# Autodesk Inventor assembly: 射出機構
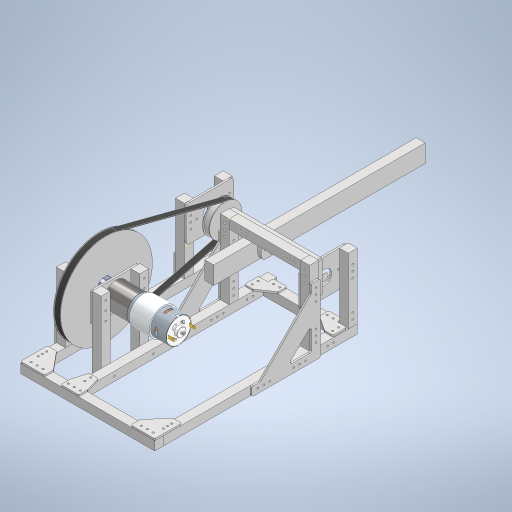
[picture p0: Inventor's stored thumbnail of the model, 512x512]
Saved by Autodesk Inventor 2023 (Build 270158000, 158)
## iProperties
Created: 2022-04-19
Part Number: 射出機構
Document SubType Name: Assembly
Designer: yuta
Author: yuta
## Documents named in this file (27)
- C:\Users\yuta\Documents\NHK\射出機構.iam
- C:\Users\yuta\Documents\NHK\RS775+gennsoku.iam
- C:\Users\yuta\Documents\NHK\射出_モーター固定1.ipt
- C:\Users\yuta\Documents\NHK\射出_type0.ipt
- C:\Users\yuta\Documents\NHK\射出_オムニ固定する.ipt
- C:\Users\yuta\Documents\NHK\射出_角柱1.ipt
- C:\Users\yuta\Documents\NHK\射出_角柱2.ipt
- C:\Users\yuta\Documents\NHK\射出_type1.ipt
- C:\Users\yuta\Documents\NHK\NHK.ipt
- C:\Users\yuta\Documents\NHK\射出_角柱3.ipt
- C:\Users\yuta\Documents\NHK\射出_角柱4.ipt
- C:\Users\yuta\Documents\NHK\射出_角柱5.ipt
- C:\Users\yuta\Documents\NHK\射出_角柱6.ipt
- C:\Users\yuta\Documents\NHK\射出_エンコーダー固定.ipt
- C:\Users\yuta\Documents\NHK\射出_固定1.ipt
- C:\Users\yuta\Documents\NHK\射出_軸.ipt
- C:\Users\yuta\Documents\NHK\射出_腕.ipt
- C:\Users\yuta\Documents\NHK\射出_角柱9.ipt
- C:\Users\yuta\Documents\NHK\射出_角柱10.ipt
- C:\Users\yuta\Documents\NHK\射出_角柱12.ipt
- C:\Users\yuta\Documents\NHK\射出_角柱11.ipt
- C:\Users\yuta\Documents\NHK\射出_受け身.ipt
- C:\Users\yuta\Documents\NHK\射出_固定2.ipt
- C:\Users\yuta\Documents\NHK\射出_固定3.ipt
- C:\Users\yuta\Documents\NHK\射出_固定4.ipt
- C:\Users\yuta\Documents\NHK\射出_固定5.ipt
- C:\Users\yuta\Documents\NHK\射出_腕固定.ipt
## Components (40 placed, 26 different names)
1. RS775+gennsoku:1 [sub-assembly] — メイト:1, メイト:2, メイト:3, メイト:4, メイト:6, メイト:16
2. 射出_モーター固定1:1 — メイト:1, メイト:2, メイト:9, メイト:10, メイト:11, メイト:12
3. 射出_オムニ固定する:1 — メイト:3, メイト:4, メイト:5
4. 射出_オムニ固定する:2 — メイト:7, メイト:8
5. 射出_type0:1 — メイト:5, メイト:6, メイト:7, メイト:8, メイト:15, メイト:17
6. 射出_角柱1:1 — メイト:9, メイト:10, メイト:13, メイト:14, メイト:47, メイト:48
7. 射出_角柱1:2 — メイト:11, メイト:12, メイト:46, メイト:48
8. 射出_角柱2:1 — メイト:13, メイト:14, フラッシュ:2, メイト:21, フラッシュ:5, フラッシュ:7, フラッシュ:8, メイト:46, メイト:47, フラッシュ:33, メイト:72, メイト:76, メイト:77
9. 射出_type1:1 — メイト:15, メイト:16, メイト:17, メイト:18, メイト:19
10. NHK:1 — メイト:18, メイト:19, メイト:35, メイト:36
11. 射出_角柱3:1 — フラッシュ:2, フラッシュ:3, メイト:20, フラッシュ:4, メイト:21, フラッシュ:5, フラッシュ:6, フラッシュ:8, メイト:22, フラッシュ:9, フラッシュ:10, メイト:67, メイト:68
12. 射出_角柱4:1 — フラッシュ:3, メイト:20, フラッシュ:4, フラッシュ:6, フラッシュ:7, メイト:37, フラッシュ:18, フラッシュ:19, メイト:53, フラッシュ:24, フラッシュ:25, メイト:58, フラッシュ:26, メイト:69, メイト:70
13. 射出_角柱5:1 — メイト:22, フラッシュ:9, フラッシュ:10, メイト:23, メイト:24, フラッシュ:11, メイト:25, フラッシュ:12, メイト:28, メイト:29, メイト:30, フラッシュ:15, フラッシュ:16, フラッシュ:17, メイト:31, メイト:66, メイト:74
14. 射出_角柱6:1 — メイト:25, メイト:26, フラッシュ:12, フラッシュ:14
15. 射出_角柱6:2 — メイト:23, メイト:24, フラッシュ:11, メイト:26, フラッシュ:13, メイト:27
16. 射出_エンコーダー固定:1 — フラッシュ:13, メイト:27, フラッシュ:14
17. 射出_固定1:2 — メイト:28, メイト:29
18. 射出_角柱6:3 — メイト:30, フラッシュ:15, フラッシュ:16, メイト:32, メイト:33, メイト:75
19. 射出_角柱6:4 — フラッシュ:17, メイト:31, メイト:32, メイト:34, フラッシュ:22
20. 射出_エンコーダー固定:2 — メイト:33, メイト:34, フラッシュ:22
21. 射出_オムニ固定する:3 — メイト:35, メイト:36
22. 射出_角柱6:5 — メイト:37, フラッシュ:18, フラッシュ:19
23. 射出_エンコーダー固定:3 — フラッシュ:23, メイト:45, メイト:55, フラッシュ:27
24. 射出_軸:1 — フラッシュ:23, メイト:45, メイト:54, メイト:79, メイト:81
25. 射出_角柱9:1 — メイト:53, フラッシュ:24, フラッシュ:25, メイト:71, メイト:73
26. 射出_腕:1 — メイト:54, メイト:55, メイト:78, メイト:80
27. 射出_角柱10:1 — メイト:58, フラッシュ:26, フラッシュ:27, メイト:59, フラッシュ:28, フラッシュ:29, メイト:62, メイト:63, メイト:64
28. 射出_角柱12:1 — メイト:59, フラッシュ:28, フラッシュ:29, メイト:60, フラッシュ:30, フラッシュ:31, メイト:61
29. 射出_角柱11:1 — メイト:60, フラッシュ:30, フラッシュ:31, メイト:65, フラッシュ:32, フラッシュ:34
30. 射出_受け身:1 — メイト:61, メイト:62, フラッシュ:34
31. 射出_固定2:2 — メイト:63, メイト:64
32. 射出_固定2:3 — メイト:65, フラッシュ:32, フラッシュ:33
33. 射出_固定3:1 — メイト:66, メイト:67
34. 射出_固定3:2 — メイト:68, メイト:69
35. 射出_固定4:1 — メイト:70, メイト:71
36. 射出_固定4:3 — メイト:72, メイト:73
37. 射出_固定1:3 — メイト:74, メイト:75
38. 射出_固定5:1 — メイト:76, メイト:77
39. 射出_腕固定:1 — メイト:78, メイト:79
40. 射出_腕固定:2 — メイト:80, メイト:81
## Relationships (99: Mate 68, Flush 31)
- メイト:1 [Mate]: RS775+gennsoku:1 ↔ 射出_モーター固定1:1
- メイト:2 [Mate]: RS775+gennsoku:1 ↔ 射出_モーター固定1:1
- メイト:3 [Mate]: RS775+gennsoku:1 ↔ 射出_オムニ固定する:1
- メイト:4 [Mate]: RS775+gennsoku:1 ↔ 射出_オムニ固定する:1
- メイト:5 [Mate]: 射出_オムニ固定する:1 ↔ 射出_type0:1
- メイト:6 [Mate]: RS775+gennsoku:1 ↔ 射出_type0:1
- メイト:7 [Mate]: 射出_オムニ固定する:2 ↔ 射出_type0:1
- メイト:8 [Mate]: 射出_オムニ固定する:2 ↔ 射出_type0:1
- メイト:9 [Mate]: 射出_モーター固定1:1 ↔ 射出_角柱1:1
- メイト:10 [Mate]: 射出_モーター固定1:1 ↔ 射出_角柱1:1
- メイト:11 [Mate]: 射出_モーター固定1:1 ↔ 射出_角柱1:2
- メイト:12 [Mate]: 射出_モーター固定1:1 ↔ 射出_角柱1:2
- メイト:13 [Mate]: 射出_角柱1:1 ↔ 射出_角柱2:1
- メイト:14 [Mate]: 射出_角柱1:1 ↔ 射出_角柱2:1
- メイト:15 [Mate]: 射出_type0:1 ↔ 射出_type1:1
- メイト:16 [Mate]: RS775+gennsoku:1 ↔ 射出_type1:1
- メイト:17 [Mate]: 射出_type0:1 ↔ 射出_type1:1
- メイト:18 [Mate]: 射出_type1:1 ↔ NHK:1
- メイト:19 [Mate]: 射出_type1:1 ↔ NHK:1
- フラッシュ:2 [Flush]: 射出_角柱2:1 ↔ 射出_角柱3:1
- フラッシュ:3 [Flush]: 射出_角柱3:1 ↔ 射出_角柱4:1
- メイト:20 [Mate]: 射出_角柱3:1 ↔ 射出_角柱4:1
- フラッシュ:4 [Flush]: 射出_角柱3:1 ↔ 射出_角柱4:1
- メイト:21 [Mate]: 射出_角柱2:1 ↔ 射出_角柱3:1
- フラッシュ:5 [Flush]: 射出_角柱2:1 ↔ 射出_角柱3:1
- フラッシュ:6 [Flush]: 射出_角柱3:1 ↔ 射出_角柱4:1
- フラッシュ:7 [Flush]: 射出_角柱2:1 ↔ 射出_角柱4:1
- フラッシュ:8 [Flush] (75 mm): 射出_角柱2:1 ↔ 射出_角柱3:1
- メイト:22 [Mate]: 射出_角柱3:1 ↔ 射出_角柱5:1
- フラッシュ:9 [Flush]: 射出_角柱3:1 ↔ 射出_角柱5:1
- フラッシュ:10 [Flush]: 射出_角柱3:1 ↔ 射出_角柱5:1
- メイト:23 [Mate]: 射出_角柱5:1 ↔ 射出_角柱6:2
- メイト:24 [Mate] (-60 mm): 射出_角柱5:1 ↔ 射出_角柱6:2
- フラッシュ:11 [Flush]: 射出_角柱5:1 ↔ 射出_角柱6:2
- メイト:25 [Mate]: 射出_角柱5:1 ↔ 射出_角柱6:1
- メイト:26 [Mate] (50 mm): 射出_角柱6:1 ↔ 射出_角柱6:2
- フラッシュ:12 [Flush]: 射出_角柱5:1 ↔ 射出_角柱6:1
- フラッシュ:13 [Flush]: 射出_角柱6:2 ↔ 射出_エンコーダー固定:1
- メイト:27 [Mate]: 射出_角柱6:2 ↔ 射出_エンコーダー固定:1
- フラッシュ:14 [Flush]: 射出_角柱6:1 ↔ 射出_エンコーダー固定:1
- メイト:28 [Mate]: 射出_角柱5:1 ↔ 射出_固定1:2
- メイト:29 [Mate]: 射出_角柱5:1 ↔ 射出_固定1:2
- メイト:30 [Mate]: 射出_角柱5:1 ↔ 射出_角柱6:3
- フラッシュ:15 [Flush]: 射出_角柱5:1 ↔ 射出_角柱6:3
- フラッシュ:16 [Flush]: 射出_角柱5:1 ↔ 射出_角柱6:3
- フラッシュ:17 [Flush]: 射出_角柱5:1 ↔ 射出_角柱6:4
- メイト:31 [Mate]: 射出_角柱5:1 ↔ 射出_角柱6:4
- メイト:32 [Mate] (50 mm): 射出_角柱6:3 ↔ 射出_角柱6:4
- メイト:33 [Mate]: 射出_角柱6:3 ↔ 射出_エンコーダー固定:2
- メイト:34 [Mate]: 射出_角柱6:4 ↔ 射出_エンコーダー固定:2
- メイト:35 [Mate]: NHK:1 ↔ 射出_オムニ固定する:3
- メイト:36 [Mate]: NHK:1 ↔ 射出_オムニ固定する:3
- メイト:37 [Mate]: 射出_角柱4:1 ↔ 射出_角柱6:5
- フラッシュ:18 [Flush]: 射出_角柱4:1 ↔ 射出_角柱6:5
- フラッシュ:19 [Flush]: 射出_角柱4:1 ↔ 射出_角柱6:5
- フラッシュ:22 [Flush]: 射出_角柱6:4 ↔ 射出_エンコーダー固定:2
- フラッシュ:23 [Flush]: 射出_エンコーダー固定:3 ↔ 射出_軸:1
- メイト:45 [Mate]: 射出_エンコーダー固定:3 ↔ 射出_軸:1
- メイト:46 [Mate]: 射出_角柱1:2 ↔ 射出_角柱2:1
- メイト:47 [Mate]: 射出_角柱1:1 ↔ 射出_角柱2:1
- メイト:48 [Mate] (50 mm): 射出_角柱1:1 ↔ 射出_角柱1:2
- メイト:53 [Mate]: 射出_角柱4:1 ↔ 射出_角柱9:1
- フラッシュ:24 [Flush] (8 mm): 射出_角柱4:1 ↔ 射出_角柱9:1
- フラッシュ:25 [Flush]: 射出_角柱4:1 ↔ 射出_角柱9:1
- メイト:54 [Mate]: 射出_軸:1 ↔ 射出_腕:1
- メイト:55 [Mate] (93 mm): 射出_エンコーダー固定:3 ↔ 射出_腕:1
- メイト:58 [Mate]: 射出_角柱4:1 ↔ 射出_角柱10:1
- フラッシュ:26 [Flush]: 射出_角柱4:1 ↔ 射出_角柱10:1
- フラッシュ:27 [Flush]: 射出_エンコーダー固定:3 ↔ 射出_角柱10:1
- メイト:59 [Mate]: 射出_角柱10:1 ↔ 射出_角柱12:1
- フラッシュ:28 [Flush]: 射出_角柱10:1 ↔ 射出_角柱12:1
- フラッシュ:29 [Flush]: 射出_角柱10:1 ↔ 射出_角柱12:1
- メイト:60 [Mate]: 射出_角柱12:1 ↔ 射出_角柱11:1
- フラッシュ:30 [Flush]: 射出_角柱12:1 ↔ 射出_角柱11:1
- フラッシュ:31 [Flush]: 射出_角柱12:1 ↔ 射出_角柱11:1
- メイト:61 [Mate]: 射出_角柱12:1 ↔ 射出_受け身:1
- メイト:62 [Mate]: 射出_角柱10:1 ↔ 射出_受け身:1
- メイト:63 [Mate]: 射出_角柱10:1 ↔ 射出_固定2:2
- メイト:64 [Mate]: 射出_角柱10:1 ↔ 射出_固定2:2
- メイト:65 [Mate]: 射出_角柱11:1 ↔ 射出_固定2:3
- フラッシュ:32 [Flush]: 射出_角柱11:1 ↔ 射出_固定2:3
- フラッシュ:33 [Flush]: 射出_角柱2:1 ↔ 射出_固定2:3
- メイト:66 [Mate]: 射出_角柱5:1 ↔ 射出_固定3:1
- メイト:67 [Mate]: 射出_角柱3:1 ↔ 射出_固定3:1
- メイト:68 [Mate]: 射出_角柱3:1 ↔ 射出_固定3:2
- メイト:69 [Mate]: 射出_角柱4:1 ↔ 射出_固定3:2
- メイト:70 [Mate]: 射出_角柱4:1 ↔ 射出_固定4:1
- メイト:71 [Mate]: 射出_角柱9:1 ↔ 射出_固定4:1
- メイト:72 [Mate]: 射出_角柱2:1 ↔ 射出_固定4:3
- メイト:73 [Mate]: 射出_角柱9:1 ↔ 射出_固定4:3
- メイト:74 [Mate]: 射出_角柱5:1 ↔ 射出_固定1:3
- メイト:75 [Mate]: 射出_角柱6:3 ↔ 射出_固定1:3
- メイト:76 [Mate]: 射出_角柱2:1 ↔ 射出_固定5:1
- メイト:77 [Mate]: 射出_角柱2:1 ↔ 射出_固定5:1
- メイト:78 [Mate]: 射出_腕:1 ↔ 射出_腕固定:1
- メイト:79 [Mate]: 射出_軸:1 ↔ 射出_腕固定:1
- メイト:80 [Mate]: 射出_腕:1 ↔ 射出_腕固定:2
- メイト:81 [Mate]: 射出_軸:1 ↔ 射出_腕固定:2
- フラッシュ:34 [Flush]: 射出_角柱11:1 ↔ 射出_受け身:1
